# Autodesk Inventor assembly: 0005-10-04 Y axis and extruder
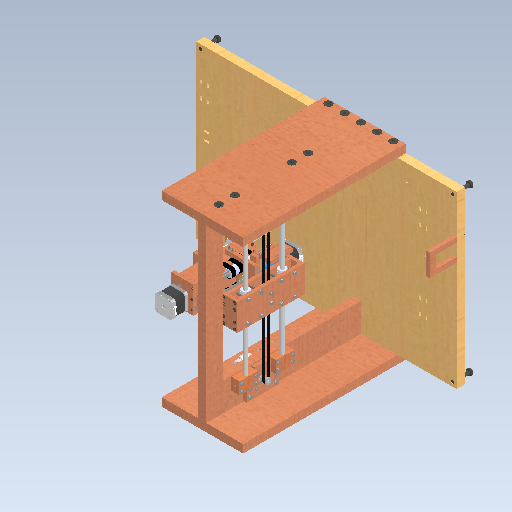
[picture p0: Inventor's stored thumbnail of the model, 512x512]
Saved by Autodesk Inventor 2020 (Build 240168000, 168)
## iProperties
Created: 2020-12-18
Part Number: 0005-10-04 Y axis and extruder
Document SubType Name: Assembly
Designer: Iulian Bors
Mass: 1667.27 g
Surface Area: 5280.79 cm^2
Volume: 1127.03 cm^3
Density: 1.47935 g/cm^3
Author: Iulian Bors
Subject: 10-04
## iProperties of the stored document Part 1.ipt
Created: 2020-12-18
Part Number: Part 1
Material: Generic
Document SubType Name: Modeling
Designer: Iulian Bors
Density: 1 g/cm^3
Appearance: Default
Mass: 0.27605 g
Surface Area: 6.48852 cm^2
Volume: 0.27605 cm^3
Author: Iulian Bors
Revision Number: NONE
## iProperties of the stored document Part 2.ipt
Created: 2020-12-18
Part Number: Part 2
Material: Generic
Document SubType Name: Modeling
Designer: Iulian Bors
Density: 1 g/cm^3
Appearance: Default
Mass: 0.0253291 g
Surface Area: 2.0565 cm^2
Volume: 0.0253291 cm^3
Author: Iulian Bors
Revision Number: NONE
## iProperties of the stored document Needle.iam
Created: 2020-01-23
Part Number: Needle
Document SubType Name: Assembly
Designer: Iulian Bors
Mass: 0.301379 g
Surface Area: 8.54503 cm^2
Volume: 0.301379 cm^3
Density: 1 g/cm^3
Title: /vol/tmp/translate-4006329005178005204/5e293bbb2de6b7156cc2e2d4.step
## Documents named in this file (42)
- Z:\I.A.B\Proiecte\0005 I.A.B 3d 2.0 Imprimanta aracet\10 Mecanic\0005-10-04 Z axis and extruder.iam
- Z:\I.A.B\Proiecte\0005 I.A.B 3d 2.0 Imprimanta aracet\10 Mecanic\Seringa\body 20ml_Défaut.ipt
- Z:\I.A.B\Proiecte\0005 I.A.B 3d 2.0 Imprimanta aracet\10 Mecanic\Seringa\Plunger Assembly_Défaut.iam
- **Z:\I.A.B\Proiecte\0005 I.A.B 3d 2.0 Imprimanta aracet\10 Mecanic\0005-10-04 Z axis and extruder.iam*LocalDocs*xAaaaqeaaAaaaaaaaAaaaq3zaLd*Needle.iam
- Z:\I.A.B\Proiecte\0005 I.A.B 3d 2.0 Imprimanta aracet\10 Mecanic\0005-10-003 Actionare seringa.ipt
- Z:\I.A.B\Proiecte\0005 I.A.B 3d 2.0 Imprimanta aracet\10 Mecanic\0005-10-004 Actionare 2 seringa.ipt
- Z:\I.A.B\Proiecte\0005 I.A.B 3d 2.0 Imprimanta aracet\10 Mecanic\0005-10-1004 Piulita.ipt
- Z:\I.A.B\Proiecte\0005 I.A.B 3d 2.0 Imprimanta aracet\10 Mecanic\0005-10-10-1003 LeadScrew 8mm x 2mmPitch.ipt
- Z:\I.A.B\Proiecte\0005 I.A.B 3d 2.0 Imprimanta aracet\10 Mecanic\0005-10-1005 ISO 1224-1 - 10 - 8 x 22 x 7.ipt
- Z:\I.A.B\Proiecte\0005 I.A.B 3d 2.0 Imprimanta aracet\10 Mecanic\0005-10-005.ipt
- Z:\I.A.B\Proiecte\0005 I.A.B 3d 2.0 Imprimanta aracet\10 Mecanic\0005-10-006 Capac rulment.ipt
- Z:\I.A.B\Proiecte\0005 I.A.B 3d 2.0 Imprimanta aracet\10 Mecanic\0005-10-1002  Hub.ipt
- Z:\I.A.B\Proiecte\0005 I.A.B 3d 2.0 Imprimanta aracet\10 Mecanic\0005-10-1001 NEMA17 - Motor de passo.ipt
- Z:\I.A.B\Proiecte\0005 I.A.B 3d 2.0 Imprimanta aracet\10 Mecanic\0005-10-007Suport nema.ipt
- Z:\I.A.B\Proiecte\0005 I.A.B 3d 2.0 Imprimanta aracet\10 Mecanic\0005-10-008.ipt
- Z:\I.A.B\Proiecte\0005 I.A.B 3d 2.0 Imprimanta aracet\10 Mecanic\0005-10-009.ipt
- Z:\I.A.B\Proiecte\0005 I.A.B 3d 2.0 Imprimanta aracet\10 Mecanic\0005-10-010.ipt
- Z:\I.A.B\Proiecte\0005 I.A.B 3d 2.0 Imprimanta aracet\10 Mecanic\0005-10-1006 Bara rectificata.ipt
- Z:\I.A.B\Proiecte\0005 I.A.B 3d 2.0 Imprimanta aracet\10 Mecanic\0005-10-1009 LM10uu.ipt
- Z:\I.A.B\Proiecte\0005 I.A.B 3d 2.0 Imprimanta aracet\10 Mecanic\0005-10-002 Suport1 Seringa.ipt
- Z:\I.A.B\Proiecte\0005 I.A.B 3d 2.0 Imprimanta aracet\10 Mecanic\0005-10-016.ipt
- Z:\I.A.B\Proiecte\0005 I.A.B 3d 2.0 Imprimanta aracet\10 Mecanic\0005-10-021 suport senzor z.ipt
- Z:\I.A.B\Proiecte\0005 I.A.B 3d 2.0 Imprimanta aracet\10 Mecanic\0005-10-1000 LM8.ipt
- Z:\I.A.B\Proiecte\0005 I.A.B 3d 2.0 Imprimanta aracet\10 Mecanic\0005-10-1018 tija 8.ipt
- Z:\I.A.B\Proiecte\0005 I.A.B 3d 2.0 Imprimanta aracet\10 Mecanic\Surub M3 40 mm.iam
- Z:\I.A.B\Proiecte\0005 I.A.B 3d 2.0 Imprimanta aracet\10 Mecanic\0005-10-1020 ISO 7089 - 3 - 140 HV(1).ipt
- Z:\I.A.B\Proiecte\0005 I.A.B 3d 2.0 Imprimanta aracet\10 Mecanic\0005-10-1032.ipt
- Z:\I.A.B\Proiecte\0005 I.A.B 3d 2.0 Imprimanta aracet\10 Mecanic\Surub M3 25.iam
- Z:\I.A.B\Proiecte\0005 I.A.B 3d 2.0 Imprimanta aracet\10 Mecanic\0005-10-1021 ISO 4032 - M3 - ISO.ipt
- Z:\I.A.B\Proiecte\0005 I.A.B 3d 2.0 Imprimanta aracet\10 Mecanic\Colier.ipt
- Z:\I.A.B\Proiecte\0005 I.A.B 3d 2.0 Imprimanta aracet\10 Mecanic\0005-10-1043 M3 x 25.ipt
- Z:\I.A.B\Proiecte\0005 I.A.B 3d 2.0 Imprimanta aracet\10 Mecanic\0005-10-1033 DIN 914 - M5 x 10.ipt
- Z:\I.A.B\Proiecte\0005 I.A.B 3d 2.0 Imprimanta aracet\10 Mecanic\0005-10-01 Cadru_Shrinkwrap_1.ipt
- Z:\I.A.B\Proiecte\0005 I.A.B 3d 2.0 Imprimanta aracet\10 Mecanic\0005-10-02 X axis_Shrinkwrap_1.ipt
- Z:\I.A.B\Proiecte\0005 I.A.B 3d 2.0 Imprimanta aracet\10 Mecanic\0005-10-1052 ISO 7050 - ST 3.5 x 16 - C - Z.ipt
- Z:\I.A.B\Proiecte\0005 I.A.B 3d 2.0 Imprimanta aracet\10 Mecanic\0005-10-1045ISO 7050 - ST 3.5 x 22 - C - Z.ipt
- Z:\I.A.B\Proiecte\0005 I.A.B 3d 2.0 Imprimanta aracet\10 Mecanic\0005-10-029 Activator Senzor Z.ipt
- **Z:\I.A.B\Proiecte\0005 I.A.B 3d 2.0 Imprimanta aracet\0005-00-00 Ansamblu_General.iam*LocalDocs*xAaaaaecaAaaaaaaaAaaaqfy1Od*Part 1.ipt
- **Z:\I.A.B\Proiecte\0005 I.A.B 3d 2.0 Imprimanta aracet\0005-00-00 Ansamblu_General.iam*LocalDocs*xAaaaa4baAaaaaaaaAaaaq4bsZa*Part 2.ipt
- **Z:\I.A.B\Proiecte\0005 I.A.B 3d 2.0 Imprimanta aracet\10 Mecanic\0005-10-04 Z axis and extruder.iam*LocalDocs*xAaaaa4baAaaaaaaaAaaaq4bsZa*Part 2.ipt
- **Z:\I.A.B\Proiecte\0005 I.A.B 3d 2.0 Imprimanta aracet\10 Mecanic\0005-10-04 Z axis and extruder.iam*LocalDocs*xAaaaaecaAaaaaaaaAaaaqfy1Od*Part 1.ipt
- Z:\I.A.B\Proiecte\0005 I.A.B 3d 2.0 Imprimanta aracet\10 Mecanic\Seringa\21-gauge-needle-1.snapshot.2\Needle.step
## Components (128 placed, 40 different names)
1. Needle.iam:1 [sub-assembly] — Insert:14
2. 0005-10-10-1003 LeadScrew 8mm x 2mmPitch.ipt:2 — Insert:2, Insert:4, Mate:61, Mate:118
3. 0005-10-1005 ISO 1224-1 - 10 - 8 x 22 x 7.ipt:3 — Insert:2, Mate:15, Insert:3
4. 0005-10-005.ipt:4 — Mate:15, Mate:16, Flush:4, Mate:17, Flush:76, Flush:7, Mate:50, Mate:51, Angle:9, Mate:59, Mate:61, Flush:35, Mate:137, Mate:138, Mate:142, Insert:67, Insert:68, Insert:111, Insert:112, Insert:113
5. 0005-10-006 Capac rulment.ipt:5 — Insert:3, Insert:62, Insert:63, Insert:64, Mate:142, Mate:143
6. 0005-10-1002  Hub.ipt:6 — Insert:4, Insert:5
7. 0005-10-1001 NEMA17 - Motor de passo.ipt:7 — Insert:5, Angle:14
8. 0005-10-008.ipt:8 — Mate:16, Flush:4, Flush:11, Mate:21, Angle:11, Mate:158, Mate:159, Insert:79, Insert:80, Insert:98, Insert:99
9. 0005-10-008.ipt:9 — Mate:17, Flush:7, Mate:119, Flush:64, Angle:16, Mate:157, Insert:81, Insert:82, Insert:100, Insert:101
10. 0005-10-016.ipt:10 — Flush:76, Mate:19, Mate:20, Flush:18, Flush:35, Flush:63, Insert:102, Insert:103
11. 0005-10-009.ipt:11 — Mate:19, Flush:11, Flush:18, Flush:63, Flush:65, Angle:15, Mate:157, Mate:158, Insert:83, Insert:84
12. 0005-10-010.ipt:12 — Mate:20, Mate:21, Insert:7, Mate:35, Mate:37, Mate:103, Insert:26, Insert:27, Mate:147, Mate:150, Mate:153, Mate:155, Mate:159, Mate:161, Flush:81
13. 0005-10-1004 Piulita.ipt:13 — Mate:35, Mate:36, Insert:115
14. 0005-10-1009 LM10uu.ipt:14 — Insert:7, Mate:26, Flush:57, Mate:145, Mate:146, Flush:80
15. 0005-10-1006 Bara rectificata.ipt:15 — Mate:26, Insert:41
16. 0005-10-1006 Bara rectificata.ipt:16 — Mate:103, Mate:104, Insert:42
17. 0005-10-10-1003 LeadScrew 8mm x 2mmPitch.ipt:17 — Mate:33, Mate:36, Mate:37, Insert:37, Insert:38
18. 0005-10-1002  Hub.ipt:18 — Mate:33
19. 0005-10-1001 NEMA17 - Motor de passo.ipt:19 — Insert:37, Mate:139, Angle:13
20. 0005-10-006 Capac rulment.ipt:20 — Insert:39, Mate:141
21. 0005-10-1005 ISO 1224-1 - 10 - 8 x 22 x 7.ipt:21 — Insert:38, Insert:39
22. 0005-10-1004 Piulita.ipt:22 — Insert:13, Mate:140, Insert:72
23. body 20ml_Défaut.ipt:23 — Mate:50, Mate:51, Angle:9, Mate:52, Insert:14
24. Plunger Assembly_Défaut.iam:24 [sub-assembly] — Mate:52, Mate:53
25. 0005-10-003 Actionare seringa.ipt:25 — Insert:13, Mate:53, Angle:11, Mate:117, Mate:118, Mate:121, Mate:140, Insert:65, Insert:66, Mate:160, Flush:77, Flush:78, Insert:104, Insert:107
26. 0005-10-004 Actionare 2 seringa.ipt:26 — Mate:160, Flush:77, Flush:78
27. 0005-10-002 Suport1 Seringa.ipt:27 — Mate:59, Mate:137, Mate:138
28. 0005-10-021 suport senzor z.ipt:28 — Mate:144, Flush:79
29. 0005-10-1009 LM10uu.ipt:29 — Mate:104, Flush:57, Mate:151, Flush:71, Mate:152
30. 0005-10-1000 LM8.ipt:30 — Mate:117, Mate:120
31. 0005-10-007Suport nema.ipt:31 — Mate:119, Flush:64, Flush:65, Flush:66, Angle:14, Insert:55, Insert:56, Insert:57, Insert:108, Insert:109, Insert:110
32. 0005-10-1018 tija 8.ipt:32 — Mate:120, Mate:121, Flush:66
33. Surub M3 40 mm.iam:33 [sub-assembly] — Insert:43
34. 0005-10-1009 LM10uu.ipt:34 — Insert:27, Mate:148, Flush:68, Mate:149
35. 0005-10-1009 LM10uu.ipt:35 — Insert:26, Mate:154, Mate:156, Flush:74
36. 0005-10-01 Cadru_Shrinkwrap_1.ipt:36 — Insert:40
37. 0005-10-02 X axis_Shrinkwrap_1.ipt:37 — Insert:40, Angle:12, Insert:41, Insert:42, Mate:139, Angle:13, Insert:43, Insert:44, Insert:45, Insert:46, Insert:58, Insert:59, Insert:60, Insert:61, Mate:144, Insert:94, Insert:95, Insert:96, Insert:97, Flush:79
38. Surub M3 40 mm.iam:38 [sub-assembly] — Insert:44, Mate:141
39. Surub M3 40 mm.iam:39 [sub-assembly] — Insert:45
40. Surub M3 40 mm.iam:40 [sub-assembly] — Insert:46
41. 0005-10-1032.ipt:41
42. 0005-10-1020 ISO 7089 - 3 - 140 HV(1).ipt:42 — Insert:55
43. 0005-10-1032.ipt:43
44. 0005-10-1020 ISO 7089 - 3 - 140 HV(1).ipt:44 — Insert:58
45. 0005-10-1032.ipt:45
46. 0005-10-1020 ISO 7089 - 3 - 140 HV(1).ipt:46 — Insert:57
47. 0005-10-1032.ipt:47
48. 0005-10-1020 ISO 7089 - 3 - 140 HV(1).ipt:48 — Insert:61
49. 0005-10-1032.ipt:49
50. 0005-10-1020 ISO 7089 - 3 - 140 HV(1).ipt:50 — Insert:59
51. 0005-10-1032.ipt:51
52. 0005-10-1020 ISO 7089 - 3 - 140 HV(1).ipt:52 — Insert:60
53. 0005-10-1032.ipt:53
54. 0005-10-1020 ISO 7089 - 3 - 140 HV(1).ipt:54 — Insert:56
55. Surub M3 40 mm.iam:55 [sub-assembly] — Insert:64
56. Surub M3 40 mm.iam:56 [sub-assembly] — Insert:63
57. Surub M3 40 mm.iam:57 [sub-assembly] — Insert:62
58. Surub M3 40 mm.iam:58 [sub-assembly] — Mate:143
59. Surub M3 25.iam:59 [sub-assembly] — Insert:65
60. Surub M3 25.iam:60 [sub-assembly] — Insert:66
61. Surub M3 25.iam:61 [sub-assembly] — Insert:67
62. Surub M3 25.iam:62 [sub-assembly] — Insert:68
63. Colier.ipt:79 — Mate:145, Angle:15, Flush:67, Flush:80
64. Colier.ipt:80 — Mate:146, Mate:147, Flush:67, Flush:69, Flush:70
65. Colier.ipt:81 — Mate:148, Flush:68, Flush:69
66. Colier.ipt:82 — Mate:149, Mate:150, Flush:70
67. Colier.ipt:83 — Mate:151, Angle:16, Flush:71, Flush:72
68. Colier.ipt:84 — Mate:152, Mate:153, Flush:72, Flush:73
69. Colier.ipt:85 — Mate:154, Mate:155, Flush:73, Flush:75
70. Colier.ipt:86 — Mate:156, Flush:74, Flush:75
71. 0005-10-1052 ISO 7050 - ST 3.5 x 16 - C - Z.ipt:93 — Insert:82
72. 0005-10-1052 ISO 7050 - ST 3.5 x 16 - C - Z.ipt:94 — Insert:81
73. 0005-10-1052 ISO 7050 - ST 3.5 x 16 - C - Z.ipt:95 — Insert:80
74. 0005-10-1052 ISO 7050 - ST 3.5 x 16 - C - Z.ipt:96 — Insert:79
75. 0005-10-1043 M3 x 25.ipt:97 — Insert:86, Insert:99
76. 0005-10-1021 ISO 4032 - M3 - ISO.ipt:98 — Insert:86
77. 0005-10-1020 ISO 7089 - 3 - 140 HV(1).ipt:99
78. 0005-10-1043 M3 x 25.ipt:100 — Insert:98
79. 0005-10-1021 ISO 4032 - M3 - ISO.ipt:101
80. 0005-10-1043 M3 x 25.ipt:102 — Insert:101
81. 0005-10-1021 ISO 4032 - M3 - ISO.ipt:103
82. 0005-10-1043 M3 x 25.ipt:104 — Insert:100
83. 0005-10-1021 ISO 4032 - M3 - ISO.ipt:105
84. 0005-10-1033 DIN 914 - M5 x 10.ipt:106 — Insert:94
85. 0005-10-1033 DIN 914 - M5 x 10.ipt:107 — Insert:95
86. 0005-10-1033 DIN 914 - M5 x 10.ipt:108 — Insert:96
87. 0005-10-1033 DIN 914 - M5 x 10.ipt:109 — Insert:97
88. 0005-10-1042.ipt:114 — Insert:102
89. 0005-10-1042.ipt:115 — Insert:103
90. ISO 7089 3:19 — Insert:104, Insert:105
91. ISO 7089 3:20 — Insert:105
92. ISO 7089 3:21 — Insert:106
93. ISO 7089 3:22 — Insert:106, Insert:107
94. ISO 7050 - C-Z ST 3.5 x 22 - C - Z:26 — Insert:113
95. ISO 7050 - C-Z ST 3.5 x 22 - C - Z:27 — Insert:110
96. ISO 7050 - C-Z ST 3.5 x 22 - C - Z:28 — Insert:108
97. ISO 7050 - C-Z ST 3.5 x 22 - C - Z:29 — Insert:112
98. ISO 7050 - C-Z ST 3.5 x 22 - C - Z:30 — Insert:111
99. ISO 7050 - C-Z ST 3.5 x 22 - C - Z:31 — Insert:109
100. 0005-10-029 Activator Senzor Z:1 — Mate:161, Flush:81
101. 0005-10-1032.ipt:63 — Insert:70
102. 0005-10-1020 ISO 7089 - 3 - 140 HV(1).ipt:64 — Insert:72
103. 0005-10-1021 ISO 4032 - M3 - ISO.ipt:65 — Insert:70, Insert:71
104. 0005-10-1020 ISO 7089 - 3 - 140 HV(1).ipt:66 — Insert:71
105. 0005-10-1032.ipt:67
106. 0005-10-1020 ISO 7089 - 3 - 140 HV(1).ipt:68
107. 0005-10-1021 ISO 4032 - M3 - ISO.ipt:69
108. 0005-10-1020 ISO 7089 - 3 - 140 HV(1).ipt:70
109. 0005-10-1032.ipt:71
110. 0005-10-1020 ISO 7089 - 3 - 140 HV(1).ipt:72
111. 0005-10-1021 ISO 4032 - M3 - ISO.ipt:73
112. 0005-10-1020 ISO 7089 - 3 - 140 HV(1).ipt:74
113. 0005-10-1032.ipt:75
114. 0005-10-1020 ISO 7089 - 3 - 140 HV(1).ipt:76
115. 0005-10-1021 ISO 4032 - M3 - ISO.ipt:77
116. 0005-10-1020 ISO 7089 - 3 - 140 HV(1).ipt:78
117. 0005-10-1042.ipt:111 — Insert:84
118. 0005-10-1042.ipt:110 — Insert:83
119. ISO 7050 - C-Z ST 3.5 x 22 - C - Z:22
120. ISO 7050 - C-Z ST 3.5 x 22 - C - Z:23
121. DIN 7984 M3 x 16:13 — Insert:115
122. ISO 4032 M3:9
123. DIN 7984 M3 x 16:14
124. ISO 4032 M3:10
125. DIN 7984 M3 x 16:15
126. ISO 4032 M3:11
127. DIN 7984 M3 x 16:16
128. ISO 4032 M3:12
## Component patterns: (4 elements, first: 0005-10-1032.ipt:63 + 0005-10-1020 ISO 7089 - 3 - 140 HV(1).ipt:64 + 0005-10-1021 ISO 4032 - M3 - ISO.ipt:65 + 0005-10-1020 ISO 7089 - 3 - 140 HV(1).ipt:66), (2 elements, first: 0005-10-1042.ipt:111 + 0005-10-1042.ipt:110), (4 elements, first: DIN 7984 M3 x 16:13 + ISO 4032 M3:9)
## Relationships (159: Insert 78, Mate 49, Flush 25, Angle 7)
- Insert:2: 0005-10-10-1003 LeadScrew 8mm x 2mmPitch.ipt:2 ↔ 0005-10-1005 ISO 1224-1 - 10 - 8 x 22 x 7.ipt:3
- Mate:15: 0005-10-1005 ISO 1224-1 - 10 - 8 x 22 x 7.ipt:3 ↔ 0005-10-005.ipt:4
- Insert:3: 0005-10-1005 ISO 1224-1 - 10 - 8 x 22 x 7.ipt:3 ↔ 0005-10-006 Capac rulment.ipt:5
- Insert:4: 0005-10-10-1003 LeadScrew 8mm x 2mmPitch.ipt:2 ↔ 0005-10-1002  Hub.ipt:6
- Insert:5 (5 mm): 0005-10-1002  Hub.ipt:6 ↔ 0005-10-1001 NEMA17 - Motor de passo.ipt:7
- Mate:16: 0005-10-005.ipt:4 ↔ 0005-10-008.ipt:8
- Flush:4: 0005-10-005.ipt:4 ↔ 0005-10-008.ipt:8
- Mate:17: 0005-10-005.ipt:4 ↔ 0005-10-008.ipt:9
- Flush:76: 0005-10-005.ipt:4 ↔ 0005-10-016.ipt:10
- Flush:7: 0005-10-005.ipt:4 ↔ 0005-10-008.ipt:9
- Mate:19 (8 mm): 0005-10-016.ipt:10 ↔ 0005-10-009.ipt:11
- Flush:11: 0005-10-008.ipt:8 ↔ 0005-10-009.ipt:11
- Mate:20: 0005-10-016.ipt:10 ↔ 0005-10-010.ipt:12
- Mate:21: 0005-10-008.ipt:8 ↔ 0005-10-010.ipt:12
- Insert:7: 0005-10-010.ipt:12 ↔ 0005-10-1009 LM10uu.ipt:14
- Mate:26: 0005-10-1009 LM10uu.ipt:14 ↔ 0005-10-1006 Bara rectificata.ipt:15
- [Insert] (5 mm): 0005-10-1002  Hub.ipt:18 ↔ 0005-10-1001 NEMA17 - Motor de passo.ipt:19
- Mate:33: 0005-10-10-1003 LeadScrew 8mm x 2mmPitch.ipt:17 ↔ 0005-10-1002  Hub.ipt:18
- Mate:35: 0005-10-010.ipt:12 ↔ 0005-10-1004 Piulita.ipt:13
- Mate:36: 0005-10-1004 Piulita.ipt:13 ↔ 0005-10-10-1003 LeadScrew 8mm x 2mmPitch.ipt:17
- Mate:37: 0005-10-010.ipt:12 ↔ 0005-10-10-1003 LeadScrew 8mm x 2mmPitch.ipt:17
- Flush:18: 0005-10-016.ipt:10 ↔ 0005-10-009.ipt:11
- Mate:50: 0005-10-005.ipt:4 ↔ body 20ml_Défaut.ipt:23
- Mate:51: 0005-10-005.ipt:4 ↔ body 20ml_Défaut.ipt:23
- Angle:9 (0 deg): 0005-10-005.ipt:4 ↔ body 20ml_Défaut.ipt:23
- Mate:52: body 20ml_Défaut.ipt:23 ↔ Plunger Assembly_Défaut.iam:24
- Insert:13: 0005-10-1004 Piulita.ipt:22 ↔ 0005-10-003 Actionare seringa.ipt:25
- Mate:53: Plunger Assembly_Défaut.iam:24 ↔ 0005-10-003 Actionare seringa.ipt:25
- Insert:14 (-5 mm): Needle.iam:1 ↔ body 20ml_Défaut.ipt:23
- Angle:11 (0 deg): 0005-10-008.ipt:8 ↔ 0005-10-003 Actionare seringa.ipt:25
- Mate:59: 0005-10-005.ipt:4 ↔ 0005-10-002 Suport1 Seringa.ipt:27
- Mate:61: 0005-10-10-1003 LeadScrew 8mm x 2mmPitch.ipt:2 ↔ 0005-10-005.ipt:4
- Flush:35 (8 mm): 0005-10-005.ipt:4 ↔ 0005-10-016.ipt:10
- Mate:103: 0005-10-010.ipt:12 ↔ 0005-10-1006 Bara rectificata.ipt:16
- Mate:104: 0005-10-1006 Bara rectificata.ipt:16 ↔ 0005-10-1009 LM10uu.ipt:29
- Flush:57: 0005-10-1009 LM10uu.ipt:14 ↔ 0005-10-1009 LM10uu.ipt:29
- Mate:117 (-10 mm): 0005-10-003 Actionare seringa.ipt:25 ↔ 0005-10-1000 LM8.ipt:30
- Mate:118: 0005-10-10-1003 LeadScrew 8mm x 2mmPitch.ipt:2 ↔ 0005-10-003 Actionare seringa.ipt:25
- Flush:63: 0005-10-016.ipt:10 ↔ 0005-10-009.ipt:11
- Mate:119: 0005-10-008.ipt:9 ↔ 0005-10-007Suport nema.ipt:31
- Flush:64: 0005-10-008.ipt:9 ↔ 0005-10-007Suport nema.ipt:31
- Flush:65: 0005-10-009.ipt:11 ↔ 0005-10-007Suport nema.ipt:31
- Mate:120: 0005-10-1000 LM8.ipt:30 ↔ 0005-10-1018 tija 8.ipt:32
- Mate:121: 0005-10-003 Actionare seringa.ipt:25 ↔ 0005-10-1018 tija 8.ipt:32
- Flush:66: 0005-10-007Suport nema.ipt:31 ↔ 0005-10-1018 tija 8.ipt:32
- Insert:26: 0005-10-010.ipt:12 ↔ 0005-10-1009 LM10uu.ipt:35
- Insert:27: 0005-10-010.ipt:12 ↔ 0005-10-1009 LM10uu.ipt:34
- Mate:137: 0005-10-005.ipt:4 ↔ 0005-10-002 Suport1 Seringa.ipt:27
- Mate:138: 0005-10-005.ipt:4 ↔ 0005-10-002 Suport1 Seringa.ipt:27
- Insert:37: 0005-10-10-1003 LeadScrew 8mm x 2mmPitch.ipt:17 ↔ 0005-10-1001 NEMA17 - Motor de passo.ipt:19
- Insert:38: 0005-10-10-1003 LeadScrew 8mm x 2mmPitch.ipt:17 ↔ 0005-10-1005 ISO 1224-1 - 10 - 8 x 22 x 7.ipt:21
- Insert:39: 0005-10-006 Capac rulment.ipt:20 ↔ 0005-10-1005 ISO 1224-1 - 10 - 8 x 22 x 7.ipt:21
- Insert:40: 0005-10-01 Cadru_Shrinkwrap_1.ipt:36 ↔ 0005-10-02 X axis_Shrinkwrap_1.ipt:37
- Angle:12 (0 deg): 0005-10-02 X axis_Shrinkwrap_1.ipt:37
- Insert:41: 0005-10-1006 Bara rectificata.ipt:15 ↔ 0005-10-02 X axis_Shrinkwrap_1.ipt:37
- Insert:42: 0005-10-1006 Bara rectificata.ipt:16 ↔ 0005-10-02 X axis_Shrinkwrap_1.ipt:37
- Mate:139: 0005-10-1001 NEMA17 - Motor de passo.ipt:19 ↔ 0005-10-02 X axis_Shrinkwrap_1.ipt:37
- Angle:13 (0 deg): 0005-10-1001 NEMA17 - Motor de passo.ipt:19 ↔ 0005-10-02 X axis_Shrinkwrap_1.ipt:37
- Angle:14 (0 deg): 0005-10-1001 NEMA17 - Motor de passo.ipt:7 ↔ 0005-10-007Suport nema.ipt:31
- Mate:140: 0005-10-1004 Piulita.ipt:22 ↔ 0005-10-003 Actionare seringa.ipt:25
- Insert:43: Surub M3 40 mm.iam:33 ↔ 0005-10-02 X axis_Shrinkwrap_1.ipt:37
- Mate:141: 0005-10-006 Capac rulment.ipt:20 ↔ Surub M3 40 mm.iam:38
- Insert:44: 0005-10-02 X axis_Shrinkwrap_1.ipt:37 ↔ Surub M3 40 mm.iam:38
- Insert:45: 0005-10-02 X axis_Shrinkwrap_1.ipt:37 ↔ Surub M3 40 mm.iam:39
- Insert:46: 0005-10-02 X axis_Shrinkwrap_1.ipt:37 ↔ Surub M3 40 mm.iam:40
- [Insert]: 0005-10-1032.ipt:41 ↔ 0005-10-1020 ISO 7089 - 3 - 140 HV(1).ipt:42
- [Insert]: 0005-10-1032.ipt:43 ↔ 0005-10-1020 ISO 7089 - 3 - 140 HV(1).ipt:44
- [Insert]: 0005-10-1032.ipt:45 ↔ 0005-10-1020 ISO 7089 - 3 - 140 HV(1).ipt:46
- [Insert]: 0005-10-1032.ipt:47 ↔ 0005-10-1020 ISO 7089 - 3 - 140 HV(1).ipt:48
- [Insert]: 0005-10-1032.ipt:49 ↔ 0005-10-1020 ISO 7089 - 3 - 140 HV(1).ipt:50
- [Insert]: 0005-10-1032.ipt:51 ↔ 0005-10-1020 ISO 7089 - 3 - 140 HV(1).ipt:52
- [Insert]: 0005-10-1032.ipt:53 ↔ 0005-10-1020 ISO 7089 - 3 - 140 HV(1).ipt:54
- Insert:55: 0005-10-007Suport nema.ipt:31 ↔ 0005-10-1020 ISO 7089 - 3 - 140 HV(1).ipt:42
- Insert:56: 0005-10-007Suport nema.ipt:31 ↔ 0005-10-1020 ISO 7089 - 3 - 140 HV(1).ipt:54
- Insert:57: 0005-10-007Suport nema.ipt:31 ↔ 0005-10-1020 ISO 7089 - 3 - 140 HV(1).ipt:46
- Insert:58: 0005-10-02 X axis_Shrinkwrap_1.ipt:37 ↔ 0005-10-1020 ISO 7089 - 3 - 140 HV(1).ipt:44
- Insert:59: 0005-10-02 X axis_Shrinkwrap_1.ipt:37 ↔ 0005-10-1020 ISO 7089 - 3 - 140 HV(1).ipt:50
- Insert:60: 0005-10-02 X axis_Shrinkwrap_1.ipt:37 ↔ 0005-10-1020 ISO 7089 - 3 - 140 HV(1).ipt:52
- Insert:61: 0005-10-02 X axis_Shrinkwrap_1.ipt:37 ↔ 0005-10-1020 ISO 7089 - 3 - 140 HV(1).ipt:48
- Insert:62: 0005-10-006 Capac rulment.ipt:5 ↔ Surub M3 40 mm.iam:57
- Insert:63: 0005-10-006 Capac rulment.ipt:5 ↔ Surub M3 40 mm.iam:56
- Insert:64: 0005-10-006 Capac rulment.ipt:5 ↔ Surub M3 40 mm.iam:55
- Mate:142: 0005-10-005.ipt:4 ↔ 0005-10-006 Capac rulment.ipt:5
- Mate:143: 0005-10-006 Capac rulment.ipt:5 ↔ Surub M3 40 mm.iam:58
- Insert:65: 0005-10-003 Actionare seringa.ipt:25 ↔ Surub M3 25.iam:59
- Insert:66: 0005-10-003 Actionare seringa.ipt:25 ↔ Surub M3 25.iam:60
- Insert:67: 0005-10-005.ipt:4 ↔ Surub M3 25.iam:61
- Insert:68: 0005-10-005.ipt:4 ↔ Surub M3 25.iam:62
- Mate:144: 0005-10-021 suport senzor z.ipt:28 ↔ 0005-10-02 X axis_Shrinkwrap_1.ipt:37
- [Insert]: 0005-10-1032.ipt:63 ↔ 0005-10-1020 ISO 7089 - 3 - 140 HV(1).ipt:64
- Insert:70: 0005-10-1032.ipt:63 ↔ 0005-10-1021 ISO 4032 - M3 - ISO.ipt:65
- Insert:71: 0005-10-1021 ISO 4032 - M3 - ISO.ipt:65 ↔ 0005-10-1020 ISO 7089 - 3 - 140 HV(1).ipt:66
- Insert:72: 0005-10-1004 Piulita.ipt:22 ↔ 0005-10-1020 ISO 7089 - 3 - 140 HV(1).ipt:64
- Mate:145: 0005-10-1009 LM10uu.ipt:14 ↔ Colier.ipt:79
- Angle:15 (180 deg): 0005-10-009.ipt:11 ↔ Colier.ipt:79
- Mate:146: 0005-10-1009 LM10uu.ipt:14 ↔ Colier.ipt:80
- Mate:147: 0005-10-010.ipt:12 ↔ Colier.ipt:80
- Flush:67: Colier.ipt:79 ↔ Colier.ipt:80
- Mate:148: 0005-10-1009 LM10uu.ipt:34 ↔ Colier.ipt:81
- Flush:68: 0005-10-1009 LM10uu.ipt:34 ↔ Colier.ipt:81
- Flush:69: Colier.ipt:80 ↔ Colier.ipt:81
- Mate:149: 0005-10-1009 LM10uu.ipt:34 ↔ Colier.ipt:82
- Mate:150: 0005-10-010.ipt:12 ↔ Colier.ipt:82
- Flush:70: Colier.ipt:80 ↔ Colier.ipt:82
- Mate:151: 0005-10-1009 LM10uu.ipt:29 ↔ Colier.ipt:83
- Angle:16 (0 deg): 0005-10-008.ipt:9 ↔ Colier.ipt:83
- Flush:71: 0005-10-1009 LM10uu.ipt:29 ↔ Colier.ipt:83
- Mate:152: 0005-10-1009 LM10uu.ipt:29 ↔ Colier.ipt:84
- Mate:153: 0005-10-010.ipt:12 ↔ Colier.ipt:84
- Flush:72: Colier.ipt:83 ↔ Colier.ipt:84
- Mate:154: 0005-10-1009 LM10uu.ipt:35 ↔ Colier.ipt:85
- Mate:155: 0005-10-010.ipt:12 ↔ Colier.ipt:85
- Flush:73: Colier.ipt:84 ↔ Colier.ipt:85
- Mate:156: 0005-10-1009 LM10uu.ipt:35 ↔ Colier.ipt:86
- Flush:74: 0005-10-1009 LM10uu.ipt:35 ↔ Colier.ipt:86
- Flush:75: Colier.ipt:85 ↔ Colier.ipt:86
- Mate:157: 0005-10-008.ipt:9 ↔ 0005-10-009.ipt:11
- Mate:158: 0005-10-008.ipt:8 ↔ 0005-10-009.ipt:11
- Mate:159: 0005-10-008.ipt:8 ↔ 0005-10-010.ipt:12
- Insert:79: 0005-10-008.ipt:8 ↔ 0005-10-1052 ISO 7050 - ST 3.5 x 16 - C - Z.ipt:96
- Insert:80: 0005-10-008.ipt:8 ↔ 0005-10-1052 ISO 7050 - ST 3.5 x 16 - C - Z.ipt:95
- Insert:81: 0005-10-008.ipt:9 ↔ 0005-10-1052 ISO 7050 - ST 3.5 x 16 - C - Z.ipt:94
- Insert:82: 0005-10-008.ipt:9 ↔ 0005-10-1052 ISO 7050 - ST 3.5 x 16 - C - Z.ipt:93
- Insert:83: 0005-10-009.ipt:11 ↔ 0005-10-1042.ipt:110
- Insert:84: 0005-10-009.ipt:11 ↔ 0005-10-1042.ipt:111
- [Insert]: 0005-10-1021 ISO 4032 - M3 - ISO.ipt:98 ↔ 0005-10-1020 ISO 7089 - 3 - 140 HV(1).ipt:99
- Insert:86 (4 mm): 0005-10-1043 M3 x 25.ipt:97 ↔ 0005-10-1021 ISO 4032 - M3 - ISO.ipt:98
- [Insert] (4 mm): 0005-10-1043 M3 x 25.ipt:100 ↔ 0005-10-1021 ISO 4032 - M3 - ISO.ipt:101
- [Insert] (4 mm): 0005-10-1043 M3 x 25.ipt:102 ↔ 0005-10-1021 ISO 4032 - M3 - ISO.ipt:103
- [Insert] (4 mm): 0005-10-1043 M3 x 25.ipt:104 ↔ 0005-10-1021 ISO 4032 - M3 - ISO.ipt:105
- Insert:94 (-5 mm): 0005-10-02 X axis_Shrinkwrap_1.ipt:37 ↔ 0005-10-1033 DIN 914 - M5 x 10.ipt:106
- Insert:95 (-5 mm): 0005-10-02 X axis_Shrinkwrap_1.ipt:37 ↔ 0005-10-1033 DIN 914 - M5 x 10.ipt:107
- Insert:96 (-5 mm): 0005-10-02 X axis_Shrinkwrap_1.ipt:37 ↔ 0005-10-1033 DIN 914 - M5 x 10.ipt:108
- Insert:97 (-5 mm): 0005-10-02 X axis_Shrinkwrap_1.ipt:37 ↔ 0005-10-1033 DIN 914 - M5 x 10.ipt:109
- Insert:98: 0005-10-008.ipt:8 ↔ 0005-10-1043 M3 x 25.ipt:100
- Insert:99: 0005-10-008.ipt:8 ↔ 0005-10-1043 M3 x 25.ipt:97
- Insert:100: 0005-10-008.ipt:9 ↔ 0005-10-1043 M3 x 25.ipt:104
- Insert:101: 0005-10-008.ipt:9 ↔ 0005-10-1043 M3 x 25.ipt:102
- Mate:160 (1 mm): 0005-10-003 Actionare seringa.ipt:25 ↔ 0005-10-004 Actionare 2 seringa.ipt:26
- Flush:77: 0005-10-003 Actionare seringa.ipt:25 ↔ 0005-10-004 Actionare 2 seringa.ipt:26
- Flush:78: 0005-10-003 Actionare seringa.ipt:25 ↔ 0005-10-004 Actionare 2 seringa.ipt:26
- Flush:79 (-10 mm): 0005-10-021 suport senzor z.ipt:28 ↔ 0005-10-02 X axis_Shrinkwrap_1.ipt:37
- Flush:80: 0005-10-1009 LM10uu.ipt:14 ↔ Colier.ipt:79
- Insert:102: 0005-10-016.ipt:10 ↔ 0005-10-1042.ipt:114
- Insert:103: 0005-10-016.ipt:10 ↔ 0005-10-1042.ipt:115
- Insert:104: 0005-10-003 Actionare seringa.ipt:25 ↔ ISO 7089 3:19
- Insert:105: ISO 7089 3:19 ↔ ISO 7089 3:20
- Insert:106: ISO 7089 3:21 ↔ ISO 7089 3:22
- Insert:107: 0005-10-003 Actionare seringa.ipt:25 ↔ ISO 7089 3:22
- Insert:108: 0005-10-007Suport nema.ipt:31 ↔ ISO 7050 - C-Z ST 3.5 x 22 - C - Z:28
- Insert:109: 0005-10-007Suport nema.ipt:31 ↔ ISO 7050 - C-Z ST 3.5 x 22 - C - Z:31
- Insert:110: 0005-10-007Suport nema.ipt:31 ↔ ISO 7050 - C-Z ST 3.5 x 22 - C - Z:27
- Insert:111: 0005-10-005.ipt:4 ↔ ISO 7050 - C-Z ST 3.5 x 22 - C - Z:30
- Insert:112: 0005-10-005.ipt:4 ↔ ISO 7050 - C-Z ST 3.5 x 22 - C - Z:29
- Insert:113: 0005-10-005.ipt:4 ↔ ISO 7050 - C-Z ST 3.5 x 22 - C - Z:26
- [Insert]: DIN 7984 M3 x 16:13 ↔ ISO 4032 M3:9
- Insert:115: 0005-10-1004 Piulita.ipt:13 ↔ DIN 7984 M3 x 16:13
- Mate:161: 0005-10-010.ipt:12 ↔ 0005-10-029 Activator Senzor Z:1
- Flush:81 (-12 mm): 0005-10-010.ipt:12 ↔ 0005-10-029 Activator Senzor Z:1
## Named parameters: d64_d31 = 5 mm, d387_d441 = 0 mm, d389_d441 = 0 mm, d390_d441 = 0 mm, d391_d441 = 0 mm, d392_d441 = 0 mm, d393_d441 = 0 mm, d412_d390_d441 = 0 mm, d460_d458 = 4 mm, d461_d458 = 4 mm, d462_d458 = 4 mm, d499_d413 = 0 mm
